# Autodesk Inventor assembly: Stewart-Body-KST215MG
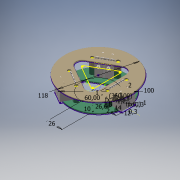
[picture p0: Inventor's stored thumbnail of the model, 180x180]
Saved by Autodesk Inventor 2018.2 (Build 222227000, 227)
## iProperties
Created: 2018-02-25
Part Number: Stewart-Body-KST215MG
Material: Generisch
Document SubType Name: Assembly
Designer: JochenAlt
Author: JochenAlt
## Documents named in this file (4)
- D:\Projects\Donna\CAD\KST DS215MG\Stewart-Body-KST215MG.iam
- D:\Projects\Donna\CAD\KST DS215MG\Stewart-Body.ipt
- D:\Projects\Donna\CAD\KST DS215MG\Servo-KST-DS215MG.ipt
- D:\Projects\Donna\CAD\KST DS215MG\Ball-Joint-male.ipt
## Components (13 placed, 3 different names)
1. Stewart-Plate:1 — Passend:3, Passend:22, Passend:23, Passend:24, Passend:25, Passend:26, Passend:27, Passend:28, Passend:29, Passend:30, Passend:31, Passend:32, Passend:33, Passend:38, Passend:39, Passend:40, Passend:41, Passend:42, Passend:43, Passend:44, Passend:45, Passend:46, Passend:47, Passend:48, Passend:49, Passend:50, Passend:51, Passend:52, Passend:53, Passend:54, Passend:55, Passend:56, Passend:57, Passend:58
2. Servo-KST-DS215MG:1 — Passend:49, Passend:51, Passend:53
3. Servo-KST-DS215MG:2 — Passend:50, Passend:52, Passend:54
4. Servo-KST-DS215MG:5 — Passend:48, Passend:56, Passend:57
5. Servo-KST-DS215MG:6 — Passend:47, Passend:55, Passend:58
6. ball joint:1 — Passend:22, Passend:28
7. ball joint:2 — Passend:23, Passend:29
8. ball joint:3 — Passend:24, Passend:33
9. ball joint:4 — Passend:25, Passend:32
10. ball joint:5 — Passend:26, Passend:31
11. ball joint:6 — Passend:27, Passend:30
12. Servo-KST-DS215MG:7 — Passend:43, Passend:44, Passend:46
13. Servo-KST-DS215MG:8 — Passend:41, Passend:42, Passend:45
## Relationships (34: Mate 34)
- Passend:3 [Mate]: Stewart-Plate:1
- Passend:22 [Mate]: Stewart-Plate:1 ↔ ball joint:1
- Passend:23 [Mate]: Stewart-Plate:1 ↔ ball joint:2
- Passend:24 [Mate]: Stewart-Plate:1 ↔ ball joint:3
- Passend:25 [Mate]: Stewart-Plate:1 ↔ ball joint:4
- Passend:26 [Mate]: Stewart-Plate:1 ↔ ball joint:5
- Passend:27 [Mate]: Stewart-Plate:1 ↔ ball joint:6
- Passend:28 [Mate]: Stewart-Plate:1 ↔ ball joint:1
- Passend:29 [Mate]: Stewart-Plate:1 ↔ ball joint:2
- Passend:30 [Mate]: Stewart-Plate:1 ↔ ball joint:6
- Passend:31 [Mate]: Stewart-Plate:1 ↔ ball joint:5
- Passend:32 [Mate]: Stewart-Plate:1 ↔ ball joint:4
- Passend:33 [Mate]: Stewart-Plate:1 ↔ ball joint:3
- Passend:38 [Mate]: Stewart-Plate:1
- Passend:39 [Mate]: Stewart-Plate:1
- Passend:40 [Mate]: Stewart-Plate:1
- Passend:41 [Mate]: Stewart-Plate:1 ↔ Servo-KST-DS215MG:8
- Passend:42 [Mate]: Stewart-Plate:1 ↔ Servo-KST-DS215MG:8
- Passend:43 [Mate]: Stewart-Plate:1 ↔ Servo-KST-DS215MG:7
- Passend:44 [Mate]: Stewart-Plate:1 ↔ Servo-KST-DS215MG:7
- Passend:45 [Mate]: Stewart-Plate:1 ↔ Servo-KST-DS215MG:8
- Passend:46 [Mate]: Stewart-Plate:1 ↔ Servo-KST-DS215MG:7
- Passend:47 [Mate]: Stewart-Plate:1 ↔ Servo-KST-DS215MG:6
- Passend:48 [Mate]: Stewart-Plate:1 ↔ Servo-KST-DS215MG:5
- Passend:49 [Mate]: Stewart-Plate:1 ↔ Servo-KST-DS215MG:1
- Passend:50 [Mate]: Stewart-Plate:1 ↔ Servo-KST-DS215MG:2
- Passend:51 [Mate]: Stewart-Plate:1 ↔ Servo-KST-DS215MG:1
- Passend:52 [Mate]: Stewart-Plate:1 ↔ Servo-KST-DS215MG:2
- Passend:53 [Mate]: Stewart-Plate:1 ↔ Servo-KST-DS215MG:1
- Passend:54 [Mate]: Stewart-Plate:1 ↔ Servo-KST-DS215MG:2
- Passend:55 [Mate]: Stewart-Plate:1 ↔ Servo-KST-DS215MG:6
- Passend:56 [Mate]: Stewart-Plate:1 ↔ Servo-KST-DS215MG:5
- Passend:57 [Mate]: Stewart-Plate:1 ↔ Servo-KST-DS215MG:5
- Passend:58 [Mate]: Stewart-Plate:1 ↔ Servo-KST-DS215MG:6
